# Autodesk Inventor assembly: Table Top and Flaps
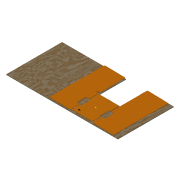
[picture p0: Inventor's stored thumbnail of the model, 180x180]
Saved by Autodesk Inventor 2016 (Build 200138000, 138)
## iProperties
Created: 2016-04-03
Part Number: Table Top and Flaps
Document SubType Name: Assembly
Designer: amycroft3
Author: amycroft3
## Documents named in this file (6)
- C:\Users\Ariana\Downloads\Capstone CAD\Capstone CAD\Table Top and Flaps.iam
- C:\Users\Ariana\Downloads\Capstone CAD\Capstone CAD\Table Top .25 in.ipt
- C:\Users\Ariana\Downloads\Capstone CAD\Capstone CAD\SideFlap.ipt
- C:\Users\Ariana\Downloads\Capstone CAD\Capstone CAD\Hinge.iam
- C:\Users\Ariana\Downloads\Capstone CAD\Capstone CAD\BottomFlap.ipt
- C:\Users\Ariana\Downloads\Capstone CAD\Capstone CAD\SideFlap2.ipt
## Components (9 placed, 5 different names)
1. Table Top .25 in:1 — Mate:16, Mate:19, Mate:20, Mate:29, Mate:30, Tangent:1, Flush:1, Mate:36, Mate:37, Flush:2, Tangent:2
2. SideFlap:2 — Mate:39, Mate:40, Mate:41, Mate:42, Flush:2
3. BottomFlap:1 — Mate:13, Mate:14, Mate:15
4. Hinge:4 [sub-assembly] — Mate:13, Mate:14, Mate:15, Mate:16, Mate:19, Mate:20
5. Hinge:5 [sub-assembly] — Mate:29, Mate:31, Angle:1, Tangent:1, Mate:35
6. Hinge:6 [sub-assembly] — Mate:30, Mate:31, Angle:1, Mate:32, Mate:33, Mate:34
7. Hinge:7 [sub-assembly] — Mate:37, Mate:38, Angle:2, Mate:39, Mate:40, Mate:41, Tangent:2
8. Hinge:8 [sub-assembly] — Mate:36, Mate:38, Angle:2, Mate:42
9. SideFlap2:1 — Mate:32, Flush:1, Mate:33, Mate:34, Mate:35
## Relationships (26: Mate 20, Angle 2, Tangent 2, Flush 2)
- Mate:13: BottomFlap:1 ↔ Hinge:4
- Mate:14: BottomFlap:1 ↔ Hinge:4
- Mate:15: BottomFlap:1 ↔ Hinge:4
- Mate:16: Table Top .25 in:1 ↔ Hinge:4
- Mate:19: Table Top .25 in:1 ↔ Hinge:4
- Mate:20: Table Top .25 in:1 ↔ Hinge:4
- Mate:29: Table Top .25 in:1 ↔ Hinge:5
- Mate:30: Table Top .25 in:1 ↔ Hinge:6
- Mate:31: Hinge:5 ↔ Hinge:6
- Angle:1 (0 deg): Hinge:5 ↔ Hinge:6
- Tangent:1 (-5.08 mm): Table Top .25 in:1 ↔ Hinge:5
- Mate:32: Hinge:6 ↔ SideFlap2:1
- Mate:33: Hinge:6 ↔ SideFlap2:1
- Mate:34: Hinge:6 ↔ SideFlap2:1
- Mate:35: Hinge:5 ↔ SideFlap2:1
- Flush:1: Table Top .25 in:1 ↔ SideFlap2:1
- Mate:36: Table Top .25 in:1 ↔ Hinge:8
- Mate:37: Table Top .25 in:1 ↔ Hinge:7
- Mate:38: Hinge:7 ↔ Hinge:8
- Angle:2 (0 deg): Hinge:7 ↔ Hinge:8
- Mate:39: SideFlap:2 ↔ Hinge:7
- Mate:40: SideFlap:2 ↔ Hinge:7
- Mate:41: SideFlap:2 ↔ Hinge:7
- Mate:42: SideFlap:2 ↔ Hinge:8
- Flush:2: Table Top .25 in:1 ↔ SideFlap:2
- Tangent:2 (-5.08 mm): Table Top .25 in:1 ↔ Hinge:7
